# Autodesk Inventor assembly: poleStand
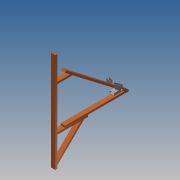
[picture p0: Inventor's stored thumbnail of the model, 180x180]
Saved by Autodesk Inventor 2013 SP2 (Build 170200200, 200)
## iProperties
Created: 2013-12-02
Part Number: poleStand
Document SubType Name: Assembly
Designer: Dave
Author: Dave
## Documents named in this file (8)
- C:\Users\Dave\Desktop\hera-cad\support\poleStand.iam
- C:\Users\Dave\Desktop\hera-cad\support\poleStandVert.ipt
- C:\Users\Dave\Desktop\hera-cad\support\poleStandHoriz1.ipt
- C:\Users\Dave\Desktop\hera-cad\support\poleStand45.ipt
- C:\Users\Dave\Desktop\hera-cad\support\poleStand37.ipt
- C:\Users\Dave\Desktop\hera-cad\support\poleStandHoriz2.ipt
- C:\Users\Dave\Desktop\hera-cad\support\poleStandHoriz3.ipt
- C:\Users\Dave\Desktop\hera-cad\support\endAssembly.iam
## Components (7 placed, 7 different names)
1. poleStandVert:1 — Insert:1, Mate:2
2. poleStand45:1 — Insert:2
3. poleStandHoriz1:1 — Insert:1, Insert:2, Mate:1
4. poleStandHoriz3:1 — Mate:2
5. poleStandHoriz2:1 — Mate:1, Insert:3
6. poleStand37:1 — Insert:3
7. endAssembly:1 [sub-assembly]
## Relationships (5: Insert 3, Mate 2)
- Insert:1: poleStandVert:1 ↔ poleStandHoriz1:1
- Insert:2: poleStand45:1 ↔ poleStandHoriz1:1
- Mate:1: poleStandHoriz1:1 ↔ poleStandHoriz2:1
- Insert:3: poleStandHoriz2:1 ↔ poleStand37:1
- Mate:2: poleStandVert:1 ↔ poleStandHoriz3:1
